# Autodesk Inventor assembly: s-assy-finger
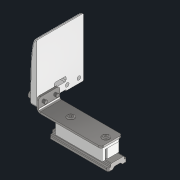
[picture p0: Inventor's stored thumbnail of the model, 180x180]
Saved by Autodesk Inventor 2021 (Build 250183000, 183)
## iProperties
Created: 2021-08-06
Part Number: s-assy-finger
Document SubType Name: Assembly
Designer: yuta0
Mass: 588.108 g
Surface Area: 2137.5 cm^2
Volume: 253.038 cm^3
Density: 2.32419 g/cm^3
Author: yuta0
## Documents named in this file (8)
- C:\Users\yuta0\Documents\GitHub\catchrobo_hardware\assy-robot\s-assy-finger.iam
- C:\Users\yuta0\Documents\GitHub\catchrobo_hardware\assy-robot\mr-20cs_1.iam
- C:\Users\yuta0\Documents\GitHub\catchrobo_hardware\assy-robot\base37.ipt
- C:\Users\yuta0\Documents\GitHub\catchrobo_hardware\assy-robot\base38.ipt
- C:\Users\yuta0\Documents\GitHub\catchrobo_hardware\assy-robot\steel_plate1.ipt
- C:\Users\yuta0\Documents\GitHub\catchrobo_hardware\assy-robot\CBSTNR3-16.ipt
- C:\Users\yuta0\Documents\GitHub\catchrobo_hardware\assy-robot\base22.ipt
- C:\Users\yuta0\Documents\GitHub\catchrobo_hardware\assy-robot\CB3-10.ipt
## Components (9 placed, 7 different names)
1. CB3-10:2 — メイト:217, メイト:218
2. CB3-10:1 — メイト:215, メイト:216
3. base22:1 — メイト:212, メイト:213, メイト:214, メイト:215, メイト:216, メイト:217, メイト:218
4. mr-20cs_1:2 [sub-assembly] — メイト:193, メイト:194
5. base37:2 — メイト:211
6. base38:2 — メイト:195, メイト:196
7. steel_plate1:2 — メイト:195, メイト:196, メイト:212, メイト:213, メイト:214
8. CBSTNR3-16:3 — メイト:193
9. CBSTNR3-16:4 — メイト:194, メイト:211
## Relationships (20: Mate 20)
- [Mate]: mr-20cs_1:2 ↔ base37:2
- [Mate]: base37:2 ↔ base38:2
- [Mate]: base37:2 ↔ base38:2
- [Mate]: base37:2 ↔ base38:2
- [Mate]: base38:2 ↔ steel_plate1:2
- [Mate]: base38:2 ↔ CBSTNR3-16:3
- [Mate]: steel_plate1:2 ↔ CBSTNR3-16:3
- [Mate]: steel_plate1:2 ↔ CBSTNR3-16:4
- メイト:193 [Mate]: mr-20cs_1:2 ↔ CBSTNR3-16:3
- メイト:194 [Mate]: mr-20cs_1:2 ↔ CBSTNR3-16:4
- メイト:195 [Mate]: base38:2 ↔ steel_plate1:2
- メイト:196 [Mate]: base38:2 ↔ steel_plate1:2
- メイト:211 [Mate]: base37:2 ↔ CBSTNR3-16:4
- メイト:212 [Mate]: base22:1 ↔ steel_plate1:2
- メイト:213 [Mate]: base22:1 ↔ steel_plate1:2
- メイト:214 [Mate]: base22:1 ↔ steel_plate1:2
- メイト:215 [Mate]: CB3-10:1 ↔ base22:1
- メイト:216 [Mate]: CB3-10:1 ↔ base22:1
- メイト:217 [Mate]: CB3-10:2 ↔ base22:1
- メイト:218 [Mate]: CB3-10:2 ↔ base22:1
## Named parameters: d270_d237 = 0 mm, d271_d238 = 0 mm, d273_d240 = 0 mm, d279_d230 = 0 mm, d289_d106 = 0 mm, d294_d139 = 0 mm, d295_d140 = 0 mm, d296_d141 = 0 mm
